# Autodesk Inventor assembly: Gripper
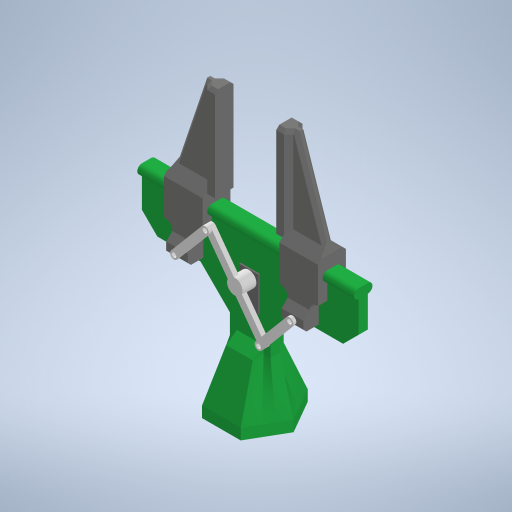
[picture p0: Inventor's stored thumbnail of the model, 512x512]
Saved by Autodesk Inventor 2023 (Build 270158000, 158)
## iProperties
Created: 2024-06-26
Part Number: Gripper
Document SubType Name: Assembly
Designer: Swoby
Author: Swoby
## Documents named in this file (6)
- C:\Users\Swoby\OneDrive\Plocha\DUM-E\V0.2\Gripper.iam
- C:\Users\Swoby\OneDrive\Plocha\DUM-E\V0.2\gripper_head.ipt
- C:\Users\Swoby\OneDrive\Plocha\DUM-E\V0.2\gripper_gripper.ipt
- C:\Users\Swoby\OneDrive\Plocha\DUM-E\V0.2\gripper_mechanism.ipt
- C:\Users\Swoby\OneDrive\Plocha\DUM-E\V0.2\gripper_mechanism2.ipt
- C:\Users\Swoby\OneDrive\Plocha\DUM-E\V0.2\Servo_small_maketa.ipt
## Components (7 placed, 5 different names)
1. gripper_head:1 — Mate:1, Mate:2, Mate:3, Mate:4, Mate:5, Mate:6, Mate:13, Mate:14, Mate:15
2. gripper_gripper:1 — Mate:1, Mate:4, Mate:10
3. gripper_gripper:2 — Mate:2, Mate:3, Mate:9
4. gripper_mechanism:1 — Mate:5, Mate:6, Mate:7, Mate:8, Mate:11, Mate:12, Mate:16, Mate:17
5. gripper_mechanism2:1 — Mate:7, Mate:10, Mate:11
6. gripper_mechanism2:2 — Mate:8, Mate:9, Mate:12
7. Servo_small_maketa:1 — Mate:13, Mate:14, Mate:15, Mate:16, Mate:17
## Relationships (17: Mate 17)
- Mate:1: gripper_head:1 ↔ gripper_gripper:1
- Mate:2: gripper_head:1 ↔ gripper_gripper:2
- Mate:3: gripper_head:1 ↔ gripper_gripper:2
- Mate:4: gripper_head:1 ↔ gripper_gripper:1
- Mate:5: gripper_head:1 ↔ gripper_mechanism:1
- Mate:6: gripper_head:1 ↔ gripper_mechanism:1
- Mate:7: gripper_mechanism:1 ↔ gripper_mechanism2:1
- Mate:8: gripper_mechanism:1 ↔ gripper_mechanism2:2
- Mate:9: gripper_gripper:2 ↔ gripper_mechanism2:2
- Mate:10: gripper_gripper:1 ↔ gripper_mechanism2:1
- Mate:11: gripper_mechanism:1 ↔ gripper_mechanism2:1
- Mate:12: gripper_mechanism:1 ↔ gripper_mechanism2:2
- Mate:13: gripper_head:1 ↔ Servo_small_maketa:1
- Mate:14: gripper_head:1 ↔ Servo_small_maketa:1
- Mate:15: gripper_head:1 ↔ Servo_small_maketa:1
- Mate:16: gripper_mechanism:1 ↔ Servo_small_maketa:1
- Mate:17: gripper_mechanism:1 ↔ Servo_small_maketa:1
